# Autodesk Inventor assembly: back-tower
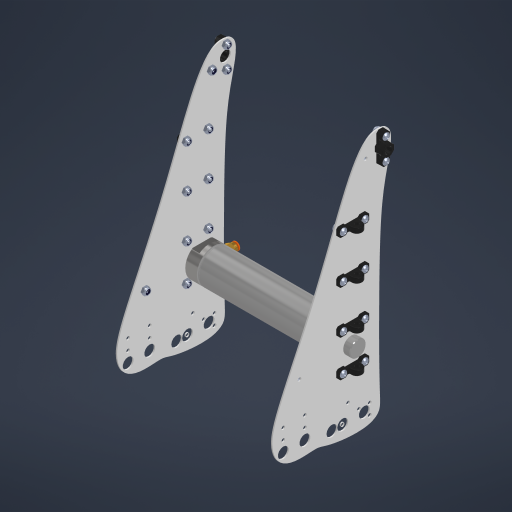
[picture p0: Inventor's stored thumbnail of the model, 512x512]
Saved by Autodesk Inventor 2023.2 (Build 272271000, 271)
## iProperties
Created: 2023-04-01
Part Number: back-tower
Document SubType Name: Assembly
Designer: Liam
Author: Liam
## Documents named in this file (10)
- D:\CAD\Robots\Spin Up\V3\back-tower.iam
- D:\CAD\Parts\custom\plastic\back-tower.ipt
- D:\CAD\Parts\standard\Motion\Bearings\HS Bearing Flat.ipt
- D:\CAD\Parts\standard\Structure\Connectors\Nut Thin Nylock.ipt
- D:\CAD\Parts\standard\Structure\Connectors\Screw Steel - Star\SScrew Star Smooth .500.ipt
- D:\CAD\Parts\standard\Structure\Connectors\Screw Steel - Star.ipt
- D:\CAD\Parts\standard\Motion\Bearings\LS Pillow Bearing Block.ipt
- D:\CAD\Parts\standard\Structure\Connectors\Screw Steel - Star\SScrew Star Smooth .375.ipt
- D:\CAD\Parts\standard\Motion\Pneumatics\Reservoir.ipt
- D:\CAD\Parts\standard\Motion\Pneumatics\Fitting for Reservoir.ipt
## Components (59 placed, 8 different names)
1. back-tower:1 — Rigid:1, Rigid:2, Rigid:6, Rigid:7, Rigid:12, Rigid:23, Rigid:24, Rigid:25, Rigid:26, Rigid:27, Rigid:28, Rigid:29, Rigid:30, Rigid:31, Rigid:32, Rigid:33, Rigid:34, Rigid:35, Rigid:58
2. back-tower:2 — Rigid:1, Rigid:3, Rigid:4, Rigid:5, Rigid:13, Rigid:14, Rigid:15, Rigid:16, Rigid:17, Rigid:18, Rigid:19, Rigid:20, Rigid:21, Rigid:22, Rigid:36, Rigid:37, Rigid:38, Rigid:39
3. HS Bearing Flat:1 — Rigid:2, Rigid:10, Rigid:11
4. HS Bearing Flat:2 — Rigid:3, Rigid:8, Rigid:9
5. Nut Thin Nylock:1 — Rigid:5
6. Nut Thin Nylock:2 — Rigid:7
7. Nut Thin Nylock:3 — Rigid:6
8. Nut Thin Nylock:4 — Rigid:4
9. SScrew Star Smooth .500:1 — Rigid:8
10. SScrew Star Smooth .500:2 — Rigid:9
11. SScrew Star Smooth .500:3 — Rigid:10
12. SScrew Star Smooth .500:4 — Rigid:11
13. Nut Thin Nylock:5 — Rigid:13
14. Nut Thin Nylock:6 — Rigid:12
15. Nut Thin Nylock:7 — Rigid:15
16. Nut Thin Nylock:8 — Rigid:14
17. Nut Thin Nylock:9 — Rigid:16
18. Nut Thin Nylock:10 — Rigid:17
19. Nut Thin Nylock:11 — Rigid:18
20. Nut Thin Nylock:12 — Rigid:19
21. Nut Thin Nylock:13 — Rigid:21
22. Nut Thin Nylock:14 — Rigid:20
23. Nut Thin Nylock:15 — Rigid:22
24. Nut Thin Nylock:16 — Rigid:23
25. Nut Thin Nylock:17 — Rigid:25
26. Nut Thin Nylock:18 — Rigid:24
27. Nut Thin Nylock:19 — Rigid:27
28. Nut Thin Nylock:20 — Rigid:26
29. Nut Thin Nylock:21 — Rigid:28
30. Nut Thin Nylock:22 — Rigid:29
31. Nut Thin Nylock:23 — Rigid:30
32. Nut Thin Nylock:24 — Rigid:31
33. LS Pillow Bearing Block:1 — Rigid:33, Rigid:42, Rigid:43
34. LS Pillow Bearing Block:2 — Rigid:34, Rigid:44, Rigid:45
35. LS Pillow Bearing Block:3 — Rigid:37, Rigid:50, Rigid:51
36. LS Pillow Bearing Block:4 — Rigid:38, Rigid:52, Rigid:53
37. LS Pillow Bearing Block:5 — Rigid:32, Rigid:40, Rigid:41
38. LS Pillow Bearing Block:6 — Rigid:35, Rigid:46, Rigid:47
39. LS Pillow Bearing Block:7 — Rigid:36, Rigid:48, Rigid:49
40. LS Pillow Bearing Block:8 — Rigid:39, Rigid:54, Rigid:55
41. SScrew Star Smooth .375:5 — Rigid:40
42. SScrew Star Smooth .375:6 — Rigid:41
43. SScrew Star Smooth .375:7 — Rigid:42
44. SScrew Star Smooth .375:8 — Rigid:43
45. SScrew Star Smooth .375:9 — Rigid:44
46. SScrew Star Smooth .375:10 — Rigid:46
47. SScrew Star Smooth .375:11 — Rigid:45
48. SScrew Star Smooth .375:12 — Rigid:47
49. SScrew Star Smooth .375:13 — Rigid:48
50. SScrew Star Smooth .375:14 — Rigid:49
51. SScrew Star Smooth .375:15 — Rigid:50
52. SScrew Star Smooth .375:16 — Rigid:51
53. SScrew Star Smooth .375:17 — Rigid:52
54. SScrew Star Smooth .375:18 — Rigid:53
55. SScrew Star Smooth .375:19 — Rigid:54
56. SScrew Star Smooth .375:20 — Rigid:55
57. Reservoir:1 — Rigid:56, Rigid:57, Rigid:58
58. Fitting for Reservoir:1 — Rigid:56
59. Fitting for Reservoir:2 — Rigid:57
## Relationships (58: WeldJoint 58)
- Rigid:1 [WeldJoint] (180.975 mm): back-tower:1 ↔ back-tower:2
- Rigid:2 [WeldJoint]: back-tower:1 ↔ HS Bearing Flat:1
- Rigid:3 [WeldJoint]: back-tower:2 ↔ HS Bearing Flat:2
- Rigid:4 [WeldJoint]: back-tower:2 ↔ Nut Thin Nylock:4
- Rigid:5 [WeldJoint]: back-tower:2 ↔ Nut Thin Nylock:1
- Rigid:6 [WeldJoint]: back-tower:1 ↔ Nut Thin Nylock:3
- Rigid:7 [WeldJoint]: back-tower:1 ↔ Nut Thin Nylock:2
- Rigid:8 [WeldJoint]: HS Bearing Flat:2 ↔ SScrew Star Smooth .500:1
- Rigid:9 [WeldJoint]: HS Bearing Flat:2 ↔ SScrew Star Smooth .500:2
- Rigid:10 [WeldJoint]: HS Bearing Flat:1 ↔ SScrew Star Smooth .500:3
- Rigid:11 [WeldJoint]: HS Bearing Flat:1 ↔ SScrew Star Smooth .500:4
- Rigid:12 [WeldJoint]: back-tower:1 ↔ Nut Thin Nylock:6
- Rigid:13 [WeldJoint]: back-tower:2 ↔ Nut Thin Nylock:5
- Rigid:14 [WeldJoint]: back-tower:2 ↔ Nut Thin Nylock:8
- Rigid:15 [WeldJoint]: back-tower:2 ↔ Nut Thin Nylock:7
- Rigid:16 [WeldJoint]: back-tower:2 ↔ Nut Thin Nylock:9
- Rigid:17 [WeldJoint]: back-tower:2 ↔ Nut Thin Nylock:10
- Rigid:18 [WeldJoint]: back-tower:2 ↔ Nut Thin Nylock:11
- Rigid:19 [WeldJoint]: back-tower:2 ↔ Nut Thin Nylock:12
- Rigid:20 [WeldJoint]: back-tower:2 ↔ Nut Thin Nylock:14
- Rigid:21 [WeldJoint]: back-tower:2 ↔ Nut Thin Nylock:13
- Rigid:22 [WeldJoint]: back-tower:2 ↔ Nut Thin Nylock:15
- Rigid:23 [WeldJoint]: back-tower:1 ↔ Nut Thin Nylock:16
- Rigid:24 [WeldJoint]: back-tower:1 ↔ Nut Thin Nylock:18
- Rigid:25 [WeldJoint]: back-tower:1 ↔ Nut Thin Nylock:17
- Rigid:26 [WeldJoint]: back-tower:1 ↔ Nut Thin Nylock:20
- Rigid:27 [WeldJoint]: back-tower:1 ↔ Nut Thin Nylock:19
- Rigid:28 [WeldJoint]: back-tower:1 ↔ Nut Thin Nylock:21
- Rigid:29 [WeldJoint]: back-tower:1 ↔ Nut Thin Nylock:22
- Rigid:30 [WeldJoint]: back-tower:1 ↔ Nut Thin Nylock:23
- Rigid:31 [WeldJoint]: back-tower:1 ↔ Nut Thin Nylock:24
- Rigid:32 [WeldJoint]: back-tower:1 ↔ LS Pillow Bearing Block:5
- Rigid:33 [WeldJoint]: back-tower:1 ↔ LS Pillow Bearing Block:1
- Rigid:34 [WeldJoint]: back-tower:1 ↔ LS Pillow Bearing Block:2
- Rigid:35 [WeldJoint]: back-tower:1 ↔ LS Pillow Bearing Block:6
- Rigid:36 [WeldJoint]: back-tower:2 ↔ LS Pillow Bearing Block:7
- Rigid:37 [WeldJoint]: back-tower:2 ↔ LS Pillow Bearing Block:3
- Rigid:38 [WeldJoint]: back-tower:2 ↔ LS Pillow Bearing Block:4
- Rigid:39 [WeldJoint]: back-tower:2 ↔ LS Pillow Bearing Block:8
- Rigid:40 [WeldJoint]: LS Pillow Bearing Block:5 ↔ SScrew Star Smooth .375:5
- Rigid:41 [WeldJoint]: LS Pillow Bearing Block:5 ↔ SScrew Star Smooth .375:6
- Rigid:42 [WeldJoint]: LS Pillow Bearing Block:1 ↔ SScrew Star Smooth .375:7
- Rigid:43 [WeldJoint]: LS Pillow Bearing Block:1 ↔ SScrew Star Smooth .375:8
- Rigid:44 [WeldJoint]: LS Pillow Bearing Block:2 ↔ SScrew Star Smooth .375:9
- Rigid:45 [WeldJoint]: LS Pillow Bearing Block:2 ↔ SScrew Star Smooth .375:11
- Rigid:46 [WeldJoint]: LS Pillow Bearing Block:6 ↔ SScrew Star Smooth .375:10
- Rigid:47 [WeldJoint]: LS Pillow Bearing Block:6 ↔ SScrew Star Smooth .375:12
- Rigid:48 [WeldJoint]: LS Pillow Bearing Block:7 ↔ SScrew Star Smooth .375:13
- Rigid:49 [WeldJoint]: LS Pillow Bearing Block:7 ↔ SScrew Star Smooth .375:14
- Rigid:50 [WeldJoint]: LS Pillow Bearing Block:3 ↔ SScrew Star Smooth .375:15
- Rigid:51 [WeldJoint]: LS Pillow Bearing Block:3 ↔ SScrew Star Smooth .375:16
- Rigid:52 [WeldJoint]: LS Pillow Bearing Block:4 ↔ SScrew Star Smooth .375:17
- Rigid:53 [WeldJoint]: LS Pillow Bearing Block:4 ↔ SScrew Star Smooth .375:18
- Rigid:54 [WeldJoint]: LS Pillow Bearing Block:8 ↔ SScrew Star Smooth .375:19
- Rigid:55 [WeldJoint]: LS Pillow Bearing Block:8 ↔ SScrew Star Smooth .375:20
- Rigid:56 [WeldJoint]: Reservoir:1 ↔ Fitting for Reservoir:1
- Rigid:57 [WeldJoint]: Reservoir:1 ↔ Fitting for Reservoir:2
- Rigid:58 [WeldJoint] (-6.35 mm): back-tower:1 ↔ Reservoir:1
